# Autodesk Inventor assembly: carriage_assemblyiam
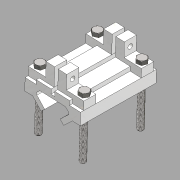
[picture p0: Inventor's stored thumbnail of the model, 180x180]
Saved by Autodesk Inventor 2020 (Build 240168000, 168)
## iProperties
Created: 2021-04-02
Part Number: carriage_assemblyiam
Document SubType Name: Assembly
Designer: griss
Author: griss
## Documents named in this file (11)
- C:\Users\griss\Documents\Inventor\CNC\y_axis_carriage\carriage_assemblyiam.iam
- C:\Users\griss\Documents\Inventor\CNC\y_axis_carriage\carriage.ipt
- C:\Users\griss\Documents\Inventor\CNC\connections\608-2RS_BALL BEARING.ipt
- C:\Users\griss\Documents\Inventor\CNC\connections\91309A640_LOW-STRENGTH ZINC-PLATED STEEL CAP SCREW.ipt
- C:\Users\griss\Documents\Inventor\CNC\connections\91309A583_LOW-STRENGTH ZINC-PLATED STEEL CAP SCREW.ipt
- C:\Users\griss\Documents\Inventor\CNC\connections\90473A030_LOW-STRENGTH STEEL HEX NUT.ipt
- C:\Users\griss\Documents\Inventor\CNC\y_axis_carriage\carriage_assemblyiam\AIP\FEA\dkbzbeqcg.fins
- C:\Users\griss\Documents\Inventor\CNC\y_axis_carriage\carriage_assemblyiam\AIP\FEA\dkbzbeqcg.fsat
- C:\Users\griss\Documents\Inventor\CNC\y_axis_carriage\carriage_assemblyiam\AIP\FEA\dkbzbeqcg.ftes
- C:\Users\griss\Documents\Inventor\CNC\y_axis_carriage\carriage_assemblyiam\AIP\FEA\dkbzbeqcg.fwiz
- C:\Users\griss\Documents\Inventor\CNC\y_axis_carriage\carriage_assemblyiam\AIP\FEA\dkbzbeqlc.fmsh
## Components (11 placed, 5 different names)
1. carriage:1 — Mate:1, Mate:2, Mate:3, Mate:4, Mate:7, Mate:8, Mate:9, Mate:10, Mate:11, Mate:14, Mate:15, Mate:16, Mate:17, Mate:18, Mate:19, Mate:20, Mate:21
2. 608-2RS_BALL BEARING:1 — Mate:8, Mate:9, Mate:12, Mate:13
3. 608-2RS_BALL BEARING:2 — Mate:10, Mate:11
4. 91309A640_LOW-STRENGTH ZINC-PLATED STEEL CAP SCREW:1 — Mate:1, Mate:19
5. 91309A640_LOW-STRENGTH ZINC-PLATED STEEL CAP SCREW:2 — Mate:2, Mate:18
6. 91309A640_LOW-STRENGTH ZINC-PLATED STEEL CAP SCREW:3 — Mate:3, Mate:20
7. 91309A640_LOW-STRENGTH ZINC-PLATED STEEL CAP SCREW:4 — Mate:4, Mate:21
8. 91309A583_LOW-STRENGTH ZINC-PLATED STEEL CAP SCREW:1 — Mate:6, Mate:12, Mate:13
9. 90473A030_LOW-STRENGTH STEEL HEX NUT:1 — Mate:6, Mate:7
10. 608-2RS_BALL BEARING:3 — Mate:14, Mate:15
11. 608-2RS_BALL BEARING:4 — Mate:16, Mate:17
## Relationships (20: Mate 20)
- Mate:1: carriage:1 ↔ 91309A640_LOW-STRENGTH ZINC-PLATED STEEL CAP SCREW:1
- Mate:2: carriage:1 ↔ 91309A640_LOW-STRENGTH ZINC-PLATED STEEL CAP SCREW:2
- Mate:3: carriage:1 ↔ 91309A640_LOW-STRENGTH ZINC-PLATED STEEL CAP SCREW:3
- Mate:4: carriage:1 ↔ 91309A640_LOW-STRENGTH ZINC-PLATED STEEL CAP SCREW:4
- Mate:6: 91309A583_LOW-STRENGTH ZINC-PLATED STEEL CAP SCREW:1 ↔ 90473A030_LOW-STRENGTH STEEL HEX NUT:1
- Mate:7: carriage:1 ↔ 90473A030_LOW-STRENGTH STEEL HEX NUT:1
- Mate:8: carriage:1 ↔ 608-2RS_BALL BEARING:1
- Mate:9: carriage:1 ↔ 608-2RS_BALL BEARING:1
- Mate:10: carriage:1 ↔ 608-2RS_BALL BEARING:2
- Mate:11: carriage:1 ↔ 608-2RS_BALL BEARING:2
- Mate:12: 608-2RS_BALL BEARING:1 ↔ 91309A583_LOW-STRENGTH ZINC-PLATED STEEL CAP SCREW:1
- Mate:13: 608-2RS_BALL BEARING:1 ↔ 91309A583_LOW-STRENGTH ZINC-PLATED STEEL CAP SCREW:1
- Mate:14: carriage:1 ↔ 608-2RS_BALL BEARING:3
- Mate:15: carriage:1 ↔ 608-2RS_BALL BEARING:3
- Mate:16: carriage:1 ↔ 608-2RS_BALL BEARING:4
- Mate:17: carriage:1 ↔ 608-2RS_BALL BEARING:4
- Mate:18: carriage:1 ↔ 91309A640_LOW-STRENGTH ZINC-PLATED STEEL CAP SCREW:2
- Mate:19: carriage:1 ↔ 91309A640_LOW-STRENGTH ZINC-PLATED STEEL CAP SCREW:1
- Mate:20: carriage:1 ↔ 91309A640_LOW-STRENGTH ZINC-PLATED STEEL CAP SCREW:3
- Mate:21: carriage:1 ↔ 91309A640_LOW-STRENGTH ZINC-PLATED STEEL CAP SCREW:4
## Named parameters: sa_0 = 4448.22
note: some values were not read from the file. Shown as the stored number, unit unknown: "sa_0".
